# Autodesk Inventor assembly: arm
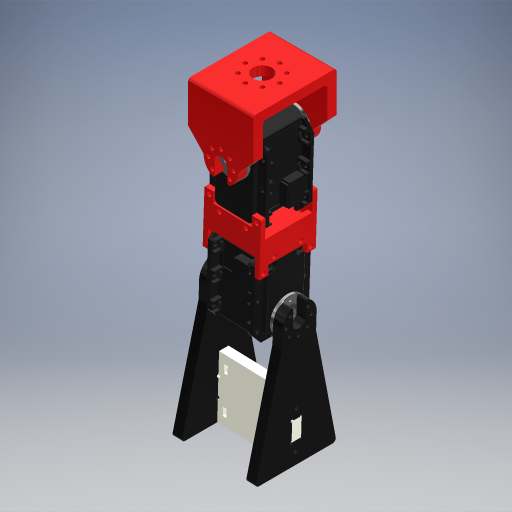
[picture p0: Inventor's stored thumbnail of the model, 512x512]
Saved by Autodesk Inventor 2024 (Build 280153000, 153)
## iProperties
Created: 2024-09-15
Part Number: arm
Document SubType Name: Assembly
Designer: msi
Author: msi
## Documents named in this file (8)
- C:\Users\msi\GITHUB\19th_intern_kgh_fight_robot\부품\Upper_body\Arm\arm_right.iam
- C:\Users\msi\GITHUB\19th_intern_kgh_fight_robot\부품\Upper_body\Arm\shoulder.ipt
- C:\Users\msi\GITHUB\19th_intern_kgh_fight_robot\부품\Upper_body\Arm\hand.ipt
- C:\Users\msi\GITHUB\19th_intern_kgh_fight_robot\부품\Upper_body\Arm\hand connection.ipt
- C:\Users\msi\GITHUB\19th_intern_kgh_fight_robot\부품\Upper_body\Arm\arm connection.ipt
- C:\Users\msi\GITHUB\19th_intern_kgh_fight_robot\부품\ROBOTIS(Inventor 2024 ver.)\다이나믹셀\MX-28T_R+idle.ipt.iam
- C:\Users\msi\GITHUB\19th_intern_kgh_fight_robot\부품\ROBOTIS(Inventor 2024 ver.)\혼\28Horn.ipt
- MX-28T_R+idle.ipt
## Components (9 placed, 6 different names)
1. shoulder:1 — 삽입:2, 삽입:3, 삽입:9
2. hand connection:1 — 삽입:12, 삽입:13, 삽입:14, 삽입:16
3. arm connection:1 — 삽입:4, 삽입:5, 삽입:18, 삽입:19
4. MX-28T_R+idle.ipt:1 [sub-assembly] — 삽입:1, 삽입:4, 삽입:5, 삽입:9
5. 28Horn:1 — 삽입:1, 삽입:2, 삽입:3
6. hand:2 — 삽입:12, 삽입:16, 삽입:20
7. hand:3 — 삽입:13, 삽입:14, 삽입:21, 삽입:22
8. MX-28T_R+idle.ipt:2 [sub-assembly] — 삽입:17, 삽입:18, 삽입:19, 삽입:20
9. 28Horn:2 — 삽입:17, 삽입:21, 삽입:22
## Relationships (16: Insert 16)
- 삽입:1 [Insert]: MX-28T_R+idle.ipt:1 ↔ 28Horn:1
- 삽입:2 [Insert]: shoulder:1 ↔ 28Horn:1
- 삽입:3 [Insert]: shoulder:1 ↔ 28Horn:1
- 삽입:4 [Insert]: arm connection:1 ↔ MX-28T_R+idle.ipt:1
- 삽입:5 [Insert]: arm connection:1 ↔ MX-28T_R+idle.ipt:1
- 삽입:9 [Insert]: shoulder:1 ↔ MX-28T_R+idle.ipt:1
- 삽입:12 [Insert]: hand connection:1 ↔ hand:2
- 삽입:13 [Insert]: hand connection:1 ↔ hand:3
- 삽입:14 [Insert]: hand connection:1 ↔ hand:3
- 삽입:16 [Insert]: hand connection:1 ↔ hand:2
- 삽입:17 [Insert]: MX-28T_R+idle.ipt:2 ↔ 28Horn:2
- 삽입:18 [Insert]: arm connection:1 ↔ MX-28T_R+idle.ipt:2
- 삽입:19 [Insert]: arm connection:1 ↔ MX-28T_R+idle.ipt:2
- 삽입:20 [Insert]: hand:2 ↔ MX-28T_R+idle.ipt:2
- 삽입:21 [Insert]: hand:3 ↔ 28Horn:2
- 삽입:22 [Insert]: hand:3 ↔ 28Horn:2
